# Autodesk Inventor assembly: Cyclone
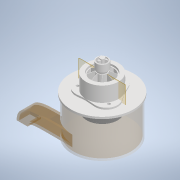
[picture p0: Inventor's stored thumbnail of the model, 180x180]
Saved by Autodesk Inventor 2020 (Build 240168000, 168)
## iProperties
Created: 2020-03-28
Part Number: Cyclone
Document SubType Name: Assembly
Designer: pengpeng
Author: pengpeng
## Documents named in this file (5)
- E:\MENG Project\Open-AMR-Hardware\Hardware\MCAD\Cyclone\Cyclone.iam
- E:\MENG Project\Open-AMR-Hardware\Hardware\MCAD\DustBin\Dust Bin.ipt
- E:\MENG Project\Open-AMR-Hardware\Hardware\MCAD\DustBin\Filter Bin.ipt
- E:\MENG Project\Open-AMR-Hardware\Hardware\MCAD\EDF\50mm_EDF.iam
- E:\MENG Project\Open-AMR-Hardware\Hardware\MCAD\DustBin\Top Lid.ipt
## Components (4 placed, 4 different names)
1. Dust Bin:1 — Mate:2, Flush:1, Mate:3, Mate:10, Mate:11, Mate:12
2. Filter Bin:1 — Mate:4, Mate:5, Mate:6
3. 50mm_EDF:1 [sub-assembly] — Mate:7, Mate:8, Mate:9
4. Top Lid:1 — Mate:4, Mate:5, Mate:6, Mate:7, Mate:8, Mate:9, Mate:10, Mate:11, Mate:12
## Relationships (12: Mate 11, Flush 1)
- Mate:2: Dust Bin:1
- Flush:1: Dust Bin:1
- Mate:3: Dust Bin:1
- Mate:4: Filter Bin:1 ↔ Top Lid:1
- Mate:5: Filter Bin:1 ↔ Top Lid:1
- Mate:6: Filter Bin:1 ↔ Top Lid:1
- Mate:7: 50mm_EDF:1 ↔ Top Lid:1
- Mate:8: 50mm_EDF:1 ↔ Top Lid:1
- Mate:9: 50mm_EDF:1 ↔ Top Lid:1
- Mate:10: Dust Bin:1 ↔ Top Lid:1
- Mate:11: Dust Bin:1 ↔ Top Lid:1
- Mate:12: Dust Bin:1 ↔ Top Lid:1
